# Autodesk Inventor assembly: CatchStructure
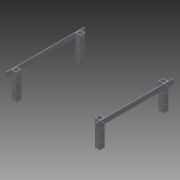
[picture p0: Inventor's stored thumbnail of the model, 180x180]
Saved by Autodesk Inventor 2013 (Build 170138000, 138)
## iProperties
Created: 2014-01-24
Part Number: CatchStructure
Document SubType Name: Assembly
Designer: Jarod
Author: Jarod
## Documents named in this file (3)
- E:\Robotics\FRC\2014\CAD\Robot\Catcher\CatchStructure.iam
- E:\Robotics\FRC\2014\CAD\Robot\Catcher\CatchPlate.ipt
- E:\Robotics\FRC\2014\CAD\Robot\Catcher\CatchSupport.ipt
## Components (6 placed, 2 different names)
1. CatchPlate:1 — Mate:9, Mate:10, Mate:11
2. CatchPlate:2 — Mate:2, Mate:3, Mate:4
3. CatchSupport:1 — Flush:3, Flush:4, Mate:8, Mate:9
4. CatchSupport:2 — Flush:1, Flush:2, Mate:1, Mate:2, Flush:5, Mate:15, Flush:6
5. CatchSupport:3 — Flush:1, Flush:2, Mate:1, Mate:3, Mate:4
6. CatchSupport:4 — Flush:3, Flush:4, Mate:8, Mate:10, Mate:11, Flush:5, Mate:15, Flush:6
## Relationships (15: Mate 9, Flush 6)
- Flush:1: CatchSupport:2 ↔ CatchSupport:3
- Flush:2: CatchSupport:2 ↔ CatchSupport:3
- Mate:1 (304.8 mm): CatchSupport:2 ↔ CatchSupport:3
- Mate:2: CatchPlate:2 ↔ CatchSupport:2
- Mate:3: CatchPlate:2 ↔ CatchSupport:3
- Mate:4: CatchPlate:2 ↔ CatchSupport:3
- Flush:3: CatchSupport:1 ↔ CatchSupport:4
- Flush:4: CatchSupport:1 ↔ CatchSupport:4
- Mate:8 (304.8 mm): CatchSupport:1 ↔ CatchSupport:4
- Mate:9: CatchPlate:1 ↔ CatchSupport:1
- Mate:10: CatchPlate:1 ↔ CatchSupport:4
- Mate:11: CatchPlate:1 ↔ CatchSupport:4
- Flush:5: CatchSupport:2 ↔ CatchSupport:4
- Mate:15 (406.4 mm): CatchSupport:2 ↔ CatchSupport:4
- Flush:6: CatchSupport:2 ↔ CatchSupport:4
